# Autodesk Inventor assembly: Pedalbox_V2_Assembly
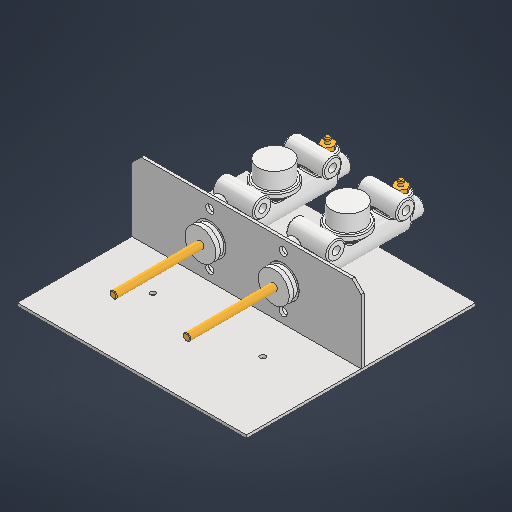
[picture p0: Inventor's stored thumbnail of the model, 512x512]
Saved by Autodesk Inventor 2026.1 (Build 301233000, 233)
## iProperties
Created: 2026-09-15
Part Number: Pedalbox_V2_Assembly
Document SubType Name: Assembly
Designer: share
Author: share
## Documents named in this file (4)
- C:\Users\share\OneDrive\Documents\Personal Projects\GOGO Kart\CAD\GOGO_KART_FSAE\Pedal Box\Pedal_Box_V2_Test\Pedalbox_V2_Assembly.iam
- C:\Users\share\OneDrive\Documents\Personal Projects\GOGO Kart\CAD\GOGO_KART_FSAE\Pedal Box\Pedal_Box_V2_Test\Pedalbox_V2_Floor.ipt
- C:\Users\share\OneDrive\Documents\Personal Projects\GOGO Kart\CAD\GOGO_KART_FSAE\Pedal Box\Pedal_Box_V2_Test\Pedalbox_V2_Vert_Rectangle.ipt
- C:\Users\share\OneDrive\Documents\Personal Projects\GOGO Kart\CAD\GOGO_KART_FSAE\Pedal Box\Pedal_Box_V2_Test\Tilton-74-Series\Tilton 74 Series\Tilton 74 Series\Tilton 74 Series.ipt
## Components (4 placed, 3 different names)
1. Pedalbox_V2_Floor:1 — Mate:1, Flush:1, Flush:2, Flush:3, Flush:4, Flush:5
2. Pedalbox_V2_Vert_Rectangle:1 — Mate:1, Flush:1, Flush:2, Insert:1, Insert:2, Insert:3
3. Tilton 74 Series:1 — Insert:1
4. Tilton 74 Series:2 — Insert:2, Insert:3
## Relationships (9: Flush 5, Insert 3, Mate 1)
- Mate:1: Pedalbox_V2_Floor:1 ↔ Pedalbox_V2_Vert_Rectangle:1
- Flush:1: Pedalbox_V2_Floor:1 ↔ Pedalbox_V2_Vert_Rectangle:1
- Flush:2 (125 mm): Pedalbox_V2_Floor:1 ↔ Pedalbox_V2_Vert_Rectangle:1
- Insert:1: Pedalbox_V2_Vert_Rectangle:1 ↔ Tilton 74 Series:1
- Flush:3: Pedalbox_V2_Floor:1
- Flush:4: Pedalbox_V2_Floor:1
- Flush:5: Pedalbox_V2_Floor:1
- Insert:2: Pedalbox_V2_Vert_Rectangle:1 ↔ Tilton 74 Series:2
- Insert:3: Pedalbox_V2_Vert_Rectangle:1 ↔ Tilton 74 Series:2
